# Autodesk Inventor assembly: final
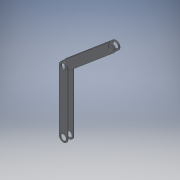
[picture p0: Inventor's stored thumbnail of the model, 180x180]
Saved by Autodesk Inventor 2019 (Build 230136000, 136)
## iProperties
Created: 2018-10-19
Part Number: final
Document SubType Name: Assembly
Designer: s-2508366
Author: s-2508366
## Documents named in this file (3)
- C:\Users\s-2508366\workspace\fbd-brachium\cad\final.iam
- C:\Users\s-2508366\workspace\fbd-brachium\cad\upper-arm-panel.ipt
- C:\Users\s-2508366\workspace\fbd-brachium\cad\forearm-panel.ipt
## Components (4 placed, 2 different names)
1. upper-arm-panel:1 — Mate:1, Mate:2, Mate:3, Mate:4, Mate:5
2. upper-arm-panel:2 — Mate:1, Mate:2, Mate:3, Mate:6, Mate:7
3. forearm-panel:1 — Mate:6, Mate:7, Mate:8
4. forearm-panel:2 — Mate:4, Mate:5, Mate:8
## Relationships (8: Mate 8)
- Mate:1: upper-arm-panel:1 ↔ upper-arm-panel:2
- Mate:2: upper-arm-panel:1 ↔ upper-arm-panel:2
- Mate:3 (25.4 mm): upper-arm-panel:1 ↔ upper-arm-panel:2
- Mate:4: upper-arm-panel:1 ↔ forearm-panel:2
- Mate:5: upper-arm-panel:1 ↔ forearm-panel:2
- Mate:6: upper-arm-panel:2 ↔ forearm-panel:1
- Mate:7: upper-arm-panel:2 ↔ forearm-panel:1
- Mate:8: forearm-panel:1 ↔ forearm-panel:2
